# Autodesk Inventor assembly: HBLTBBN45-SET_MIR
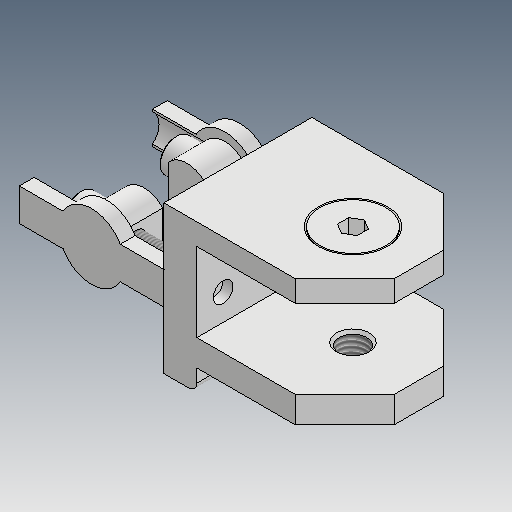
[picture p0: Inventor's stored thumbnail of the model, 512x512]
Saved by Autodesk Inventor 2020 (Build 240168000, 168)
## iProperties
Category: PARTsolutions
Company: MISUMI
Part Number: HBLTBBN45-SET_MIR
Catalog Web Link: www.cadenas.de
Description: HBLTBBN-Free Angle Brackets
Vendor: MISUMI
Document SubType Name: Assembly
Designer: magnarecta
Manufacturer: MISUMI
Mass: 55.6041 g
Surface Area: 223.171 cm^2
Volume: 55.6041 cm^3
Density: 1 g/cm^3
Title: HBLTBBN45-SET
Author: Cadenas PARTsolutions
Comments: Free Angle Brackets
PSOL_IDENT_0: {$CADENAS_DATA\23d-libs\misumi\metric\38_al_extrusions_blackets\hbltbbn_asmtab.prj},177 {VTYP=3D},{S
PSOL_IDENT_1: TYP=ASSTAB},{NB=HBLTBBN45-SET},{LINA=HBLTBBN45-SET},{NN=HBLTBBN},{DATE=08.06.2021 08:27:28},{GEOMDAT
PSOL_IDENT_2: E=21.12.2009},{VERSION=},{LINEID=100},{WBVAR=ALT1},{WBNUMERIC=}  {NB=HBLTBBN45-SET},{LINA=HBLTBBN45-
PSOL_IDENT_3: SET},{KT=DUMMY},{PN=HBLTBBN45-SET},{TP=HBLTBBN},{NO=45},{TNS=HBLTBBN45},{MATMB=A6N01SS-T5},{MATAB=41
PSOL_IDENT_4: 37 Alloy Steel},{STMB=Anodize},{STAB=Trivalent Chromate},{CS=45 Square (HFS8-45)},{A=45},{MA=6},{MAN=
PSOL_IDENT_5: 6},{N=-},{NN=0.0},{T=10},{TT1=6.5},{TT2=8.0},{W=24.0},{H=35},{H1=55},{E=29},{EN=29.0},{F=8},{FN=8.0}
PSOL_IDENT_6: ,{C=15},{CN=15},{M=10},{L=16},{MASS=116.0},{AHS=M10x16},{ALT1=-SET},{ALT1ATT= '' , 'w/o Applicable B
PSOL_IDENT_7: olt and Nut Set' , '-SET' , 'with SET (Applicable Bolt and Nut Set)'   },{UM=-},{ACB=CBM6-35},{ACBD=
PSOL_IDENT_8: 6},{ACBL=35},{ACBQ=2},{ACN=HDJFSN8-45},{ACNQ=1},{X=4},{MD=11.0},{PPATH=hbltba_asmtpl.prj},{HFSH=6.00
PSOL_IDENT_9: 0}
NB: HBLTBBN45-SET
NN: HBLTBBN
NT: Free Angle Brackets
NBSYN: $PN.
LINA: HBLTBBN45-SET
CATALOG: Misumi
PN: HBLTBBN45-SET
TNS: HBLTBBN45
MATMB: A6N01SS-T5 Aluminum Alloy
MATAB: 4137 Alloy Steel
STMB: Clear Anodizing
STAB: Trivalent Chromate Plating
CS: 45 Square (HFS8-45)
A: 45
MA: 6
T: 10
TT1: 6.5
TT2: 8
W: 24
H: 35
H1: 55
E: 29
F: 8
C: 15
M: 10
MASS: 116
AHS: M10x16
ALT1: with SET (Applicable Bolt and Nut Set)
UM: -
ACB: CBM6-35
ACBQ: 2
ACN: HDJFSN8-45
ACNQ: 1
SUPPLIER: MISUMI
ARTICLENO: HBLTBBN45-SET
BOMINFO: HBLTBBN45-SET
CREATOR: CADENAS GmbH
## Documents named in this file (5)
- D:\Documents\GitHub\Eto_Project\Hardware\Parts\MISUMI\HBLTBBN45-SET_Autodesk_Inventor_2020_20211206\AIS2020\HBLTBBN45-SET_MIR.iam
- D:\Documents\GitHub\Eto_Project\Hardware\Parts\MISUMI\HBLTBBN45-SET_Autodesk_Inventor_2020_20211206\AIS2020\HBLTBBN45-SET_b_MIR.ipt
- D:\Documents\GitHub\Eto_Project\Hardware\Parts\MISUMI\HBLTBBN45-SET_Autodesk_Inventor_2020_20211206\AIS2020\FB10-16__MIR.ipt
- D:\Documents\GitHub\Eto_Project\Hardware\Parts\MISUMI\HBLTBBN45-SET_Autodesk_Inventor_2020_20211206\AIS2020\HDJSN8-45__j_MIR.ipt
- D:\Documents\GitHub\Eto_Project\Hardware\Parts\MISUMI\HBLTBBN45-SET_Autodesk_Inventor_2020_20211206\AIS2020\CBM6-35_MIR.ipt
## Components (6 placed, 4 different names)
1. HBLTBBN45-SET_b_MIR:1 — bracket_to_screw_Z@1 <-> screw_to_nut_Z@2, screw3_Z@1 <-> screw_Z@3, screw3_1_Z@1 <-> screw_Z@4, screw1_1_Z@1 <-> bolt_Z@5, screw1_1_XY@1 <-> bolt_XY@5, screw1_2_Z@1 <-> bolt_Z@6, screw1_2_XY@1 <-> bolt_XY@6, screw1_1_YZ@1 <-> bolt_YZ@5, screw1_2_YZ@1 <-> bolt_YZ@6
2. FB10-16__MIR:1 — bracket_to_screw_Z@1 <-> screw_to_nut_Z@2
3. HDJSN8-45__j_MIR:1 — screw3_Z@1 <-> screw_Z@3
4. HDJSN8-45__j_MIR:2 — screw3_1_Z@1 <-> screw_Z@4
5. CBM6-35_MIR:1 — screw1_1_Z@1 <-> bolt_Z@5, screw1_1_XY@1 <-> bolt_XY@5, screw1_1_YZ@1 <-> bolt_YZ@5
6. CBM6-35_MIR:2 — screw1_2_Z@1 <-> bolt_Z@6, screw1_2_XY@1 <-> bolt_XY@6, screw1_2_YZ@1 <-> bolt_YZ@6
## Relationships (9: Mate 7, Angle 2)
- bracket_to_screw_Z@1 <-> screw_to_nut_Z@2 [Mate]: HBLTBBN45-SET_b_MIR:1 ↔ FB10-16__MIR:1
- screw3_Z@1 <-> screw_Z@3 [Mate]: HBLTBBN45-SET_b_MIR:1 ↔ HDJSN8-45__j_MIR:1
- screw3_1_Z@1 <-> screw_Z@4 [Mate]: HBLTBBN45-SET_b_MIR:1 ↔ HDJSN8-45__j_MIR:2
- screw1_1_Z@1 <-> bolt_Z@5 [Mate]: HBLTBBN45-SET_b_MIR:1 ↔ CBM6-35_MIR:1
- screw1_1_XY@1 <-> bolt_XY@5 [Mate]: HBLTBBN45-SET_b_MIR:1 ↔ CBM6-35_MIR:1
- screw1_2_Z@1 <-> bolt_Z@6 [Mate]: HBLTBBN45-SET_b_MIR:1 ↔ CBM6-35_MIR:2
- screw1_2_XY@1 <-> bolt_XY@6 [Mate]: HBLTBBN45-SET_b_MIR:1 ↔ CBM6-35_MIR:2
- screw1_1_YZ@1 <-> bolt_YZ@5 [Angle] (0 deg): HBLTBBN45-SET_b_MIR:1 ↔ CBM6-35_MIR:1
- screw1_2_YZ@1 <-> bolt_YZ@6 [Angle] (0 deg): HBLTBBN45-SET_b_MIR:1 ↔ CBM6-35_MIR:2
